# Autodesk Inventor assembly: 6 HiGrip with hub and double pulley
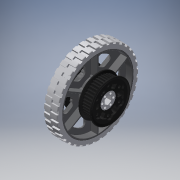
[picture p0: Inventor's stored thumbnail of the model, 180x180]
Saved by Autodesk Inventor 2017 (Build 210142000, 142)
## iProperties
Part Number: 6 HiGrip with hub and double pulley
Material: 一般
Document SubType Name: Assembly
Designer: IJA
Author: IJA
Revision Number: ANY
## Documents named in this file (6)
- D:\Works\Robot2\6 HiGrip with hub and double pulley.iam
- D:\Works\Robot2\6 HiGrip Asm Rev II.iam
- D:\Works\Robot2\42 tooth HTD Pulley half 2014.ipt
- D:\Works\Robot2\10-24 Hex Washer Rolling x 1.25_93882A213.ipt
- D:\Works\Robot2\500EX Hex Hub.ipt
- D:\Works\Robot2\am-1305 500 Hex Spacer.ipt
## Components (19 placed, 19 different names)
1. 6 HiGrip Asm Rev II_17 [sub-assembly] — 貼合:1
2. 42 tooth HTD Pulley half 2014_18
3. 42 tooth HTD Pulley half 2014_19
4. 10-24 Hex Washer Rolling x 1.25_93882A213_20
5. 10-24 Hex Washer Rolling x 1.25_93882A213_21
6. 10-24 Hex Washer Rolling x 1.25_93882A213_22
7. 10-24 Hex Washer Rolling x 1.25_93882A213_23
8. 10-24 Hex Washer Rolling x 1.25_93882A213_24
9. 10-24 Hex Washer Rolling x 1.25_93882A213_25
10. 42 tooth HTD Pulley half 2014_26
11. 42 tooth HTD Pulley half 2014_27
12. 500EX Hex Hub_28
13. 10-24 Hex Washer Rolling x 1.25_93882A213_29
14. 10-24 Hex Washer Rolling x 1.25_93882A213_30
15. 10-24 Hex Washer Rolling x 1.25_93882A213_31
16. 10-24 Hex Washer Rolling x 1.25_93882A213_32
17. 10-24 Hex Washer Rolling x 1.25_93882A213_33
18. 10-24 Hex Washer Rolling x 1.25_93882A213_34
19. am-1305 500 Hex Spacer_35 — 貼合:1
## Relationships (1: Mate 1)
- 貼合:1 [Mate]: 6 HiGrip Asm Rev II_17 ↔ am-1305 500 Hex Spacer_35
